# Autodesk Inventor assembly: 810001-X1
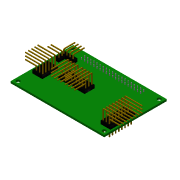
[picture p0: Inventor's stored thumbnail of the model, 180x180]
Saved by Autodesk Inventor 2015 (Build 190159000, 159)
## iProperties
Created: 2013-01-19
Part Number: 810001-X1
Document SubType Name: Assembly
Designer: davidgitz
Author: davidgitz
## Documents named in this file (5)
- C:\SharedDrive\Dropbox\FAST Robotics\Products\810001_FAST Robot Shield\CAD\810001_FAST Robot Shield\810001-X1.iam
- C:\SharedDrive\Dropbox\FAST Robotics\Products\810001_FAST Robot Shield\CAD\810001_FAST Robot Shield\MainBoard.ipt
- C:\SharedDrive\Dropbox\FAST Robotics\Products\811000_Parallax Quickstart\CAD\811000_Parallax Quickstart\702871018.ipt
- C:\SharedDrive\Dropbox\FAST Robotics\Products\810001_FAST Robot Shield\CAD\810001_FAST Robot Shield\HeaderRight3.ipt
- C:\SharedDrive\Dropbox\FAST Robotics\Products\810001_FAST Robot Shield\CAD\810001_FAST Robot Shield\HeaderRight1.ipt
## Components (29 placed, 4 different names)
1. MainBoard:1 — Mate:9, Flush:12, Flush:13, Mate:10, Flush:14, Flush:15, Flush:16, Flush:17, Flush:18, Mate:11, Flush:19, Flush:20, Mate:12, Mate:13, Flush:21, Flush:22, Flush:24, Mate:14, Flush:25, Mate:15, Flush:27
2. 702871018:1 — Mate:9, Flush:12, Flush:13
3. HeaderRight3:2 — Mate:10
4. HeaderRight3:3 — Flush:17
5. HeaderRight3:4
6. HeaderRight3:5
7. HeaderRight3:6 — Flush:18
8. HeaderRight3:1 — Mate:11, Flush:20
9. HeaderRight3:7
10. HeaderRight3:8
11. HeaderRight3:9
12. HeaderRight3:10
13. HeaderRight3:11
14. HeaderRight3:12
15. HeaderRight3:13 — Flush:19
16. HeaderRight3:14 — Mate:12, Flush:21
17. HeaderRight3:16 — Flush:22
18. HeaderRight3:17
19. HeaderRight3:18 — Flush:23
20. HeaderRight3:15 — Mate:13
21. HeaderRight3:19
22. HeaderRight3:20
23. HeaderRight3:21 — Flush:23, Flush:24
24. HeaderRight1:1 — Mate:14, Flush:25, Mate:16, Flush:26
25. HeaderRight1:2
26. HeaderRight1:3 — Mate:15
27. HeaderRight1:4
28. HeaderRight1:5 — Flush:27
29. HeaderRight1:6 — Mate:16, Flush:26
## Component patterns: GPIO5x3 (5 elements), ANA8x3 (8 elements), US4x3 (4 elements), SRV4x3 (4 elements), SERVOPOWER2x1 (2 elements), (4 elements, first: HeaderRight1:3)
## Relationships (24: Flush 16, Mate 8)
- Mate:9: MainBoard:1 ↔ 702871018:1
- Flush:12 (3.048 mm): MainBoard:1 ↔ 702871018:1
- Flush:13 (12.446 mm): MainBoard:1 ↔ 702871018:1
- Mate:10: MainBoard:1 ↔ HeaderRight3:2
- Flush:14: MainBoard:1
- Flush:15: MainBoard:1
- Flush:16: MainBoard:1
- Flush:17 (3.429 mm): MainBoard:1 ↔ HeaderRight3:3
- Flush:18 (14.351 mm): MainBoard:1 ↔ HeaderRight3:6
- Mate:11: MainBoard:1 ↔ HeaderRight3:1
- Flush:19 (1.27 mm): MainBoard:1 ↔ HeaderRight3:13
- Flush:20 (-6.35 mm): MainBoard:1 ↔ HeaderRight3:1
- Mate:12: MainBoard:1 ↔ HeaderRight3:14
- Mate:13: MainBoard:1 ↔ HeaderRight3:15
- Flush:21 (-17.78 mm): MainBoard:1 ↔ HeaderRight3:14
- Flush:22 (-21.844 mm): MainBoard:1 ↔ HeaderRight3:16
- Flush:23: HeaderRight3:18 ↔ HeaderRight3:21
- Flush:24 (29.21 mm): MainBoard:1 ↔ HeaderRight3:21
- Mate:14: MainBoard:1 ↔ HeaderRight1:1
- Flush:25 (-3.429 mm): MainBoard:1 ↔ HeaderRight1:1
- Mate:15: MainBoard:1 ↔ HeaderRight1:3
- Mate:16: HeaderRight1:1 ↔ HeaderRight1:6
- Flush:26: HeaderRight1:1 ↔ HeaderRight1:6
- Flush:27 (-10.16 mm): MainBoard:1 ↔ HeaderRight1:5
